# Autodesk Inventor assembly: Parameter
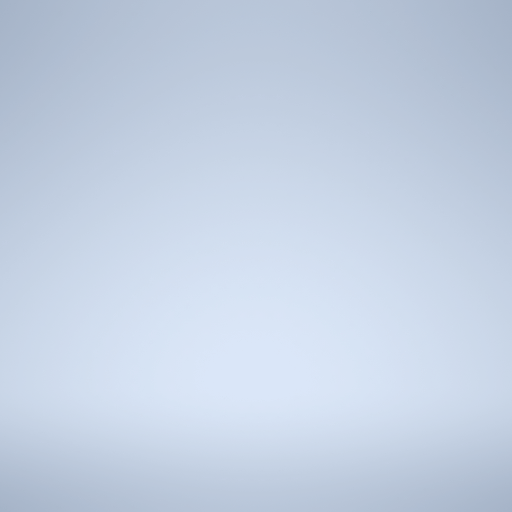
[picture p0: Inventor's stored thumbnail of the model, 512x512]
Saved by Autodesk Inventor 2025 (Build 290162010, 162A)
## iProperties
Created: 2024-11-20
Part Number: Parameter
Document SubType Name: Assembly
Designer: Admin
schrägWinkel: 1,59 grd
höheFrame: 483,000 mm
seildurchmesser: 2,000 mm
Author: Admin
## Documents named in this file (1)
- C:\Users\Admin\GIT\HDVKBM\CAD\Krandemonstrator\Parameter.iam
## Named parameters: schrägWinkel = 1.587669 deg, höheFrame = 483 mm, seildurchmesser = 2 mm
